# Autodesk Inventor assembly: Shoulder Joint Assembly
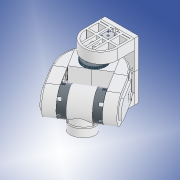
[picture p0: Inventor's stored thumbnail of the model, 180x180]
Saved by Autodesk Inventor 2017 SP1 (Build 210196100, 196)
## iProperties
Created: 2017-06-01
Part Number: Shoulder Joint Assembly
Document SubType Name: Assembly
Designer: Zach
Author: Zach
## Documents named in this file (22)
- C:\Users\Zach\Documents\GitHub\cr-laundry-robot\src\Body\Arm Assembly\Shoulder Joint Assembly\Shoulder Joint Assembly.iam
- C:\Users\Zach\Documents\GitHub\cr-laundry-robot\src\Body\Arm Assembly\Shoulder Joint Assembly\SJ002.ipt
- C:\Users\Zach\Documents\GitHub\cr-laundry-robot\src\Body\Arm Assembly\Shoulder Joint Assembly\SJ003.ipt
- C:\Users\Zach\Documents\GitHub\cr-laundry-robot\src\Body\Arm Assembly\Shoulder Joint Assembly\SJ001.ipt
- C:\Users\Zach\Documents\GitHub\cr-laundry-robot\lib\Stepper Motor - NEMA 17\NEMA17.ipt
- C:\Users\Zach\Documents\GitHub\cr-laundry-robot\src\Body\Arm Assembly\Shoulder Joint Assembly\SJ004.ipt
- C:\Users\Zach\Documents\GitHub\cr-laundry-robot\src\Body\Arm Assembly\Shoulder Joint Assembly\SJ005.ipt
- C:\Users\Zach\Documents\GitHub\cr-laundry-robot\src\Body\Arm Assembly\Shoulder Joint Assembly\SJ006.ipt
- C:\Users\Zach\Documents\GitHub\cr-laundry-robot\lib\U51105\U51105.ipt
- C:\Users\Zach\Documents\GitHub\cr-laundry-robot\lib\QS12MM250\QS12MM250.ipt
- C:\Users\Zach\Documents\GitHub\cr-laundry-robot\lib\6201RS\6201RS.ipt
- C:\Users\Zach\Documents\GitHub\cr-laundry-robot\src\Body\Arm Assembly\Shoulder Joint Assembly\SJ007.ipt
- C:\Users\Zach\Documents\GitHub\cr-laundry-robot\src\Body\Arm Assembly\Shoulder Joint Assembly\SJ008.ipt
- C:\Users\Zach\Documents\GitHub\cr-laundry-robot\src\Body\Arm Assembly\Shoulder Joint Assembly\Shoulder Joint Assembly\Design Accelerator\Spur Gears1.iam
- C:\Users\Zach\Documents\GitHub\cr-laundry-robot\src\Body\Arm Assembly\Shoulder Joint Assembly\SJ009.ipt
- C:\Users\Zach\Documents\GitHub\cr-laundry-robot\lib\Strain Wave Gearbox\StrainWaveGearbox.iam
- C:\Users\Zach\Documents\GitHub\cr-laundry-robot\lib\22x8x8mm Bearing.ipt
- C:\Users\Zach\Documents\GitHub\cr-laundry-robot\src\Body\Arm Assembly\Shoulder Joint Assembly\Shoulder Joint Assembly\Design Accelerator\Spur Gears2.iam
- C:\Users\Zach\Documents\GitHub\cr-laundry-robot\src\Body\Arm Assembly\Shoulder Joint Assembly\Shoulder Joint Assembly\Design Accelerator\Spur Gears3.iam
- C:\Users\Zach\Documents\GitHub\cr-laundry-robot\src\Body\Arm Assembly\Shoulder Joint Assembly\SJ017.ipt
- C:\Users\Zach\Documents\GitHub\cr-laundry-robot\src\Body\Arm Assembly\Shoulder Joint Assembly\Shoulder Joint Assembly\Design Accelerator\Spur Gears4.iam
- C:\Users\Zach\Documents\GitHub\cr-laundry-robot\src\Body\Arm Assembly\Shoulder Joint Assembly\SJ018.ipt
## Components (41 placed, 18 different names)
1. SJ001:1 — Mate:47, Mate:173, Mate:176, Mate:232, Mate:234, Mate:235, Mate:270, Mate:271, Mate:272, Mate:273, Mate:274, Mate:277, Mate:278, Mate:279, Mate:280, Mate:281
2. SJ001:2 — Mate:162, Mate:168, Mate:169, Mate:170, Mate:199, Mate:201, Mate:208, Mate:209, Mate:210, Mate:211, Mate:249, Mate:251, Mate:252, Mate:253, Mate:254, Mate:255, Mate:256, Mate:257, Mate:258, Mate:265, Mate:266, Mate:267, Mate:268, Mate:283, Mate:284, Mate:285
3. SJ002:1 — Mate:1, Mate:4, Mate:8, Mate:9, Mate:174, Mate:178
4. SJ002:2 — Mate:18, Mate:19, Mate:20, Mate:172
5. SJ003:1 — Mate:1, Mate:4, Mate:8, Mate:9, Mate:18, Mate:19, Mate:20, Mate:148, Mate:149, Mate:150, Mate:164, Mate:165, Mate:167, Mate:294, Mate:295
6. SJ004:1 — Mate:130, Mate:162, Mate:163, Mate:209, Mate:210, Mate:211, Mate:212, Mate:213, Mate:214
7. SJ004:2 — Mate:47, Mate:54, Mate:55, Mate:56, Mate:216, Mate:217
8. SJ005:1 — Mate:54, Mate:55, Mate:56, Mate:60, Mate:67, Mate:69, Mate:70, Mate:80, Flush:1, Mate:218
9. SJ005:2 — Mate:68, Mate:82, Mate:84, Mate:130, Mate:136, Flush:1, Mate:163, Mate:214, Mate:218
10. SJ006:2 — Mate:67, Mate:68, Mate:69, Mate:70, Mate:78, Mate:79, Mate:83
11. NEMA17:3 — Mate:148, Mate:149, Mate:150, Mate:286
12. U51105:1 — Mate:131, Mate:139, Mate:215
13. U51105:2 — Mate:78, Mate:79
14. QS12MM250:1 — Mate:80, Mate:105, Mate:117, Mate:119, Mate:120, Mate:132, Mate:134, Mate:215
15. 6201RS:1 — Mate:82, Mate:138
16. 6201RS:2 — Mate:83, Mate:84
17. SJ007:1 — Mate:121, Mate:122, Mate:123, Mate:133
18. SJ008:1 — Mate:119, Mate:125, Mate:126, Mate:127, Mate:132
19. SJ008:2 — Mate:97, Mate:98, Mate:99, Mate:105, Mate:112, Mate:117, Mate:120, Mate:121, Mate:122, Mate:123, Mate:124, Mate:131
20. NEMA17:4 — Mate:97, Mate:98, Mate:99, Mate:137
21. SJ007:2 — Mate:125, Mate:126, Mate:127, Mate:133
22. Spur Gears:1 [sub-assembly] — Mate:134, Mate:136, Mate:137, Mate:138, Mate:139
23. SJ009:1 — Mate:212, Mate:213
24. SJ009:2 — Mate:216, Mate:217
25. StrainWaveGearbox:1 [sub-assembly] — Mate:164, Mate:165, Mate:288, Mate:293, Mate:294
26. StrainWaveGearbox:2 [sub-assembly] — Mate:167, Mate:168, Mate:169, Mate:170, Mate:172
27. StrainWaveGearbox:3 [sub-assembly] — Mate:173, Mate:174, Mate:176, Mate:178
28. NEMA17:5 — Mate:199, Mate:201, Mate:208, Mate:282
29. 22x8x8mm Bearing:1 — Mate:249, Mate:252
30. 22x8x8mm Bearing:2 — Mate:251, Mate:254
31. 22x8x8mm Bearing:4 — Mate:273, Mate:274, Mate:296
32. 22x8x8mm Bearing:5 — Mate:275, Mate:276
33. NEMA17:6 — Mate:232, Mate:234, Mate:235, Mate:269
34. Spur Gears:2 [sub-assembly] — Mate:253, Mate:282, Mate:283, Mate:284, Mate:285
35. Spur Gears:3 [sub-assembly] — Mate:255, Mate:265, Mate:266, Mate:267, Mate:268
36. SJ017:1 — Mate:256, Mate:257, Mate:258
37. Spur Gears:4 [sub-assembly] — Mate:275, Mate:276, Mate:277, Mate:278, Mate:296
38. Spur Gears:5 [sub-assembly] — Mate:269, Mate:270, Mate:271, Mate:272
39. SJ017:2 — Mate:279, Mate:280, Mate:281
40. Spur Gears:6 [sub-assembly] — Mate:286, Mate:288, Mate:290, Mate:291, Mate:292, Mate:295
41. SJ018:1 — Mate:290, Mate:291, Mate:292, Mate:293
## Relationships (118: Mate 117, Flush 1)
- Mate:1: SJ002:1 ↔ SJ003:1
- Mate:4: SJ002:1 ↔ SJ003:1
- Mate:8: SJ002:1 ↔ SJ003:1
- Mate:9: SJ002:1 ↔ SJ003:1
- Mate:18: SJ002:2 ↔ SJ003:1
- Mate:19: SJ002:2 ↔ SJ003:1
- Mate:20: SJ002:2 ↔ SJ003:1
- Mate:47: SJ001:1 ↔ SJ004:2
- Mate:54: SJ004:2 ↔ SJ005:1
- Mate:55: SJ004:2 ↔ SJ005:1
- Mate:56: SJ004:2 ↔ SJ005:1
- Mate:60: SJ005:1
- Mate:67: SJ005:1 ↔ SJ006:2
- Mate:68: SJ005:2 ↔ SJ006:2
- Mate:69: SJ005:1 ↔ SJ006:2
- Mate:70: SJ005:1 ↔ SJ006:2
- Mate:78: SJ006:2 ↔ U51105:2
- Mate:79: SJ006:2 ↔ U51105:2
- Mate:80: SJ005:1 ↔ QS12MM250:1
- Mate:82: SJ005:2 ↔ 6201RS:1
- Mate:83: SJ006:2 ↔ 6201RS:2
- Mate:84: SJ005:2 ↔ 6201RS:2
- Mate:97: SJ008:2 ↔ NEMA17:4
- Mate:98: SJ008:2 ↔ NEMA17:4
- Mate:99: SJ008:2 ↔ NEMA17:4
- Mate:105: QS12MM250:1 ↔ SJ008:2
- Mate:112: SJ008:2
- Mate:117: QS12MM250:1 ↔ SJ008:2
- Mate:119: QS12MM250:1 ↔ SJ008:1
- Mate:120: QS12MM250:1 ↔ SJ008:2
- Mate:121: SJ007:1 ↔ SJ008:2
- Mate:122: SJ007:1 ↔ SJ008:2
- Mate:123: SJ007:1 ↔ SJ008:2
- Mate:124: SJ008:2
- Mate:125: SJ008:1 ↔ SJ007:2
- Mate:126: SJ008:1 ↔ SJ007:2
- Mate:127: SJ008:1 ↔ SJ007:2
- Mate:130: SJ004:1 ↔ SJ005:2
- Mate:131: U51105:1 ↔ SJ008:2
- Mate:132: QS12MM250:1 ↔ SJ008:1
- Mate:133: SJ007:1 ↔ SJ007:2
- Mate:134: QS12MM250:1 ↔ Spur Gears:1
- Mate:136: SJ005:2 ↔ Spur Gears:1
- Mate:137: NEMA17:4 ↔ Spur Gears:1
- Mate:138: 6201RS:1 ↔ Spur Gears:1
- Mate:139: U51105:1 ↔ Spur Gears:1
- Mate:148: SJ003:1 ↔ NEMA17:3
- Mate:149: SJ003:1 ↔ NEMA17:3
- Mate:150: SJ003:1 ↔ NEMA17:3
- Mate:162: SJ001:2 ↔ SJ004:1
- Flush:1: SJ005:1 ↔ SJ005:2
- Mate:163: SJ004:1 ↔ SJ005:2
- Mate:164: SJ003:1 ↔ StrainWaveGearbox:1
- Mate:165: SJ003:1 ↔ StrainWaveGearbox:1
- Mate:167: SJ003:1 ↔ StrainWaveGearbox:2
- Mate:168: SJ001:2 ↔ StrainWaveGearbox:2
- Mate:169: SJ001:2 ↔ StrainWaveGearbox:2
- Mate:170: SJ001:2 ↔ StrainWaveGearbox:2
- Mate:172: SJ002:2 ↔ StrainWaveGearbox:2
- Mate:173: SJ001:1 ↔ StrainWaveGearbox:3
- Mate:174: SJ002:1 ↔ StrainWaveGearbox:3
- Mate:176: SJ001:1 ↔ StrainWaveGearbox:3
- Mate:178: SJ002:1 ↔ StrainWaveGearbox:3
- Mate:199: SJ001:2 ↔ NEMA17:5
- Mate:201: SJ001:2 ↔ NEMA17:5
- Mate:208: SJ001:2 ↔ NEMA17:5
- Mate:209: SJ001:2 ↔ SJ004:1
- Mate:210: SJ001:2 ↔ SJ004:1
- Mate:211: SJ001:2 ↔ SJ004:1
- Mate:212: SJ004:1 ↔ SJ009:1
- Mate:213: SJ004:1 ↔ SJ009:1
- Mate:214: SJ004:1 ↔ SJ005:2
- Mate:215: U51105:1 ↔ QS12MM250:1
- Mate:216: SJ004:2 ↔ SJ009:2
- Mate:217: SJ004:2 ↔ SJ009:2
- Mate:218: SJ005:1 ↔ SJ005:2
- Mate:232: SJ001:1 ↔ NEMA17:6
- Mate:234: SJ001:1 ↔ NEMA17:6
- Mate:235: SJ001:1 ↔ NEMA17:6
- Mate:249: SJ001:2 ↔ 22x8x8mm Bearing:1
- Mate:251: SJ001:2 ↔ 22x8x8mm Bearing:2
- Mate:252: SJ001:2 ↔ 22x8x8mm Bearing:1
- Mate:253: SJ001:2 ↔ Spur Gears:2
- Mate:254: SJ001:2 ↔ 22x8x8mm Bearing:2
- Mate:255: SJ001:2 ↔ Spur Gears:3
- Mate:256: SJ001:2 ↔ SJ017:1
- Mate:257: SJ001:2 ↔ SJ017:1
- Mate:258: SJ001:2 ↔ SJ017:1
- Mate:265: SJ001:2 ↔ Spur Gears:3
- Mate:266: SJ001:2 ↔ Spur Gears:3
- Mate:267: SJ001:2 ↔ Spur Gears:3
- Mate:268: SJ001:2 ↔ Spur Gears:3
- Mate:269: NEMA17:6 ↔ Spur Gears:5
- Mate:270: SJ001:1 ↔ Spur Gears:5
- Mate:271: SJ001:1 ↔ Spur Gears:5
- Mate:272: SJ001:1 ↔ Spur Gears:5
- Mate:273: SJ001:1 ↔ 22x8x8mm Bearing:4
- Mate:274: SJ001:1 ↔ 22x8x8mm Bearing:4
- Mate:275: 22x8x8mm Bearing:5 ↔ Spur Gears:4
- Mate:276: 22x8x8mm Bearing:5 ↔ Spur Gears:4
- Mate:277: SJ001:1 ↔ Spur Gears:4
- Mate:278: SJ001:1 ↔ Spur Gears:4
- Mate:279: SJ001:1 ↔ SJ017:2
- Mate:280: SJ001:1 ↔ SJ017:2
- Mate:281: SJ001:1 ↔ SJ017:2
- Mate:282: NEMA17:5 ↔ Spur Gears:2
- Mate:283: SJ001:2 ↔ Spur Gears:2
- Mate:284: SJ001:2 ↔ Spur Gears:2
- Mate:285: SJ001:2 ↔ Spur Gears:2
- Mate:286: NEMA17:3 ↔ Spur Gears:6
- Mate:288: StrainWaveGearbox:1 ↔ Spur Gears:6
- Mate:290: Spur Gears:6 ↔ SJ018:1
- Mate:291: Spur Gears:6 ↔ SJ018:1
- Mate:292: Spur Gears:6 ↔ SJ018:1
- Mate:293: StrainWaveGearbox:1 ↔ SJ018:1
- Mate:294: SJ003:1 ↔ StrainWaveGearbox:1
- Mate:295: SJ003:1 ↔ Spur Gears:6
- Mate:296: 22x8x8mm Bearing:4 ↔ Spur Gears:4
